# Autodesk Inventor assembly: Handpumpe
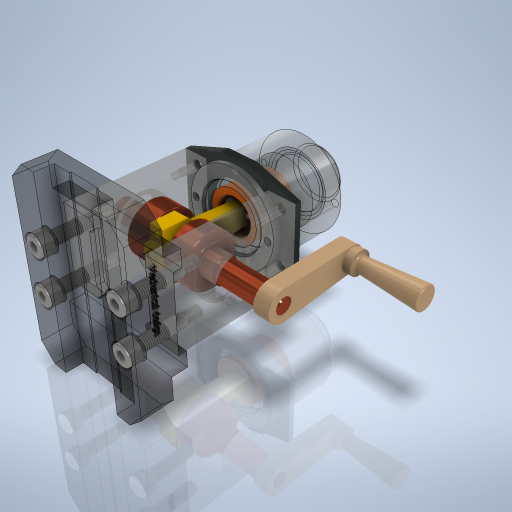
[picture p0: Inventor's stored thumbnail of the model, 512x512]
Saved by Autodesk Inventor 2024.2 (Build 282272000, 272)
## iProperties
Created: 2024-03-04
Part Number: Handpumpe
Document SubType Name: Assembly
Designer: ffogue
Author: ffogue
## Documents named in this file (14)
- C:\Users\Fabri\Documents\Inventor\Handpumpe\Handpumpe.iam
- C:\Users\Fabri\Documents\Inventor\Handpumpe\Grundplatte.ipt
- C:\Users\Fabri\Documents\Inventor\Handpumpe\Pleuel_oberteil.ipt
- C:\Users\Fabri\Documents\Inventor\Handpumpe\Pleuel_Unterteil.ipt
- C:\Users\Fabri\Documents\Inventor\Handpumpe\HAlteplatte.ipt
- C:\Users\Fabri\Documents\Inventor\Handpumpe\Lagerbock_MIR.ipt
- C:\Users\Fabri\Documents\Inventor\Handpumpe\Zylinder_laufbuechse.ipt
- C:\Users\Fabri\Documents\Inventor\Handpumpe\Kolben.ipt
- C:\Users\Fabri\Documents\Inventor\Handpumpe\Exzenterwlle.ipt
- C:\Users\Fabri\Documents\Inventor\Handpumpe\Kurbelarm.ipt
- C:\Users\Fabri\Documents\Inventor\Handpumpe\Griff.ipt
- C:\Users\Fabri\Documents\Inventor\Handpumpe\kolbenverbindung.ipt
- C:\Users\Fabri\Documents\Inventor\Handpumpe\Zylinder.ipt
- C:\Users\Fabri\Documents\Inventor\Content Center Files\R2024\de-DE\DIN 912\DIN 912 - M8 x 1,25 x 30 x 26,875.ipt
## Components (18 placed, 13 different names)
1. Grundplatte:1 — Fluchtend:1, Fluchtend:2, Fluchtend:3, Passend:1, Passend:2, Einfügen:1, Einfügen:2, Einfügen:12, Einfügen:13, Einfügen:14, Einfügen:15
2. Lagerbock_MIR:1 — Passend:1, Einfügen:1, Einfügen:6, Symmetrie:1, Einfügen:11
3. Lagerbock_MIR:2 — Passend:2, Einfügen:2, Einfügen:5, Winkel:4, Symmetrie:1
4. Kolben:1 — Einfügen:5
5. Exzenterwlle:1 — Einfügen:6, Zylindrisch:1, Motion, Einfügen:8, Passend:3, Winkel:3
6. Pleuel_oberteil:1 — Zylindrisch:1, Einfügen:7, Einfügen:10
7. Pleuel_Unterteil:1 — Einfügen:7
8. Kurbelarm:1 — Einfügen:8, Passend:3, Winkel:3, Passend:4, Einfügen:9
9. Griff:1 — Passend:4, Einfügen:9
10. Kolben:2 — Drehbar:1, Winkel:4, Zylindrisch:2, Zylindrisch:5
11. kolbenverbindung:1 — Einfügen:10, Drehbar:1
12. HAlteplatte:1 — Zylindrisch:2, Einfügen:11, Zylindrisch:3
13. Zylinder:1 — Zylindrisch:3, Zylindrisch:4
14. Zylinder_laufbuechse:1 — Zylindrisch:4, Zylindrisch:5
15. DIN 912 - ersetzt durch DIN EN ISO 4762 M8 x 30:1 — Einfügen:14
16. DIN 912 - ersetzt durch DIN EN ISO 4762 M8 x 30:2 — Einfügen:15
17. DIN 912 - ersetzt durch DIN EN ISO 4762 M8 x 30:3 — Einfügen:13
18. DIN 912 - ersetzt durch DIN EN ISO 4762 M8 x 30:4 — Einfügen:12
## Relationships (32: Insert 13, Flush 5, CylindricalJoint 5, Mate 4, Angle 3, RevoluteJoint 1, Symmetry 1)
- Fluchtend:1 [Flush]: Grundplatte:1
- Fluchtend:2 [Flush]: Grundplatte:1
- Fluchtend:3 [Flush]: Grundplatte:1
- Fluchtend:10 [Flush] (-41.5 mm)
- Passend:1 [Mate]: Grundplatte:1 ↔ Lagerbock_MIR:1
- Passend:2 [Mate]: Grundplatte:1 ↔ Lagerbock_MIR:2
- Einfügen:1 [Insert]: Grundplatte:1 ↔ Lagerbock_MIR:1
- Einfügen:2 [Insert]: Grundplatte:1 ↔ Lagerbock_MIR:2
- Einfügen:5 [Insert] (-10 mm): Lagerbock_MIR:2 ↔ Kolben:1
- Einfügen:6 [Insert] (-1 mm): Lagerbock_MIR:1 ↔ Exzenterwlle:1
- Zylindrisch:1 [CylindricalJoint]: Exzenterwlle:1 ↔ Pleuel_oberteil:1
- Einfügen:7 [Insert]: Pleuel_oberteil:1 ↔ Pleuel_Unterteil:1
- Motion [Angle] (3600 deg): Exzenterwlle:1
- Einfügen:8 [Insert] (-8.5 mm): Exzenterwlle:1 ↔ Kurbelarm:1
- Passend:3 [Mate]: Exzenterwlle:1 ↔ Kurbelarm:1
- Winkel:3 [Angle] (0 deg): Exzenterwlle:1 ↔ Kurbelarm:1
- Passend:4 [Mate]: Kurbelarm:1 ↔ Griff:1
- Einfügen:9 [Insert] (-10 mm): Kurbelarm:1 ↔ Griff:1
- Einfügen:10 [Insert] (-21.5 mm): Pleuel_oberteil:1 ↔ kolbenverbindung:1
- Drehbar:1 [RevoluteJoint] (-30 mm): Kolben:2 ↔ kolbenverbindung:1
- Winkel:4 [Angle] (180 deg): Lagerbock_MIR:2 ↔ Kolben:2
- Fluchtend:11 [Flush] (-41.5 mm)
- Symmetrie:1: Lagerbock_MIR:1 ↔ Lagerbock_MIR:2
- Zylindrisch:2 [CylindricalJoint]: Kolben:2 ↔ HAlteplatte:1
- Einfügen:11 [Insert]: Lagerbock_MIR:1 ↔ HAlteplatte:1
- Zylindrisch:3 [CylindricalJoint]: HAlteplatte:1 ↔ Zylinder:1
- Zylindrisch:4 [CylindricalJoint]: Zylinder:1 ↔ Zylinder_laufbuechse:1
- Zylindrisch:5 [CylindricalJoint]: Kolben:2 ↔ Zylinder_laufbuechse:1
- Einfügen:12 [Insert] (-28 mm): Grundplatte:1 ↔ DIN 912 - ersetzt durch DIN EN ISO 4762 M8 x 30:4
- Einfügen:13 [Insert] (-28 mm): Grundplatte:1 ↔ DIN 912 - ersetzt durch DIN EN ISO 4762 M8 x 30:3
- Einfügen:14 [Insert] (-28 mm): Grundplatte:1 ↔ DIN 912 - ersetzt durch DIN EN ISO 4762 M8 x 30:1
- Einfügen:15 [Insert] (-28 mm): Grundplatte:1 ↔ DIN 912 - ersetzt durch DIN EN ISO 4762 M8 x 30:2
